# Autodesk Inventor assembly: RailMirrorIrisLens
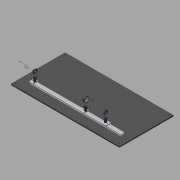
[picture p0: Inventor's stored thumbnail of the model, 180x180]
Saved by Autodesk Inventor 2018 (Build 220112000, 112)
## iProperties
Created: 2018-11-05
Part Number: RailMirrorIrisLens
Document SubType Name: Assembly
Designer: Robert Campbell
Author: Robert Campbell
## Documents named in this file (5)
- \\Mac\Home\Dropbox (UCL - SWC)\work\WorkDocs\MF_BenchOptics\CAD_files\RailMirrorIrisLens.iam
- \\Mac\Home\Dropbox (UCL - SWC)\work\WorkDocs\MF_BenchOptics\CAD_files\RailAndMirror.iam
- \\Mac\Home\Dropbox (UCL - SWC)\work\WorkDocs\MF_BenchOptics\CAD_files\R2_M-Step.ipt
- \\Mac\Home\Dropbox (UCL - SWC)\work\WorkDocs\MF_BenchOptics\CAD_files\LA1256-A-Solidworks.ipt
- \\Mac\Home\Dropbox (UCL - SWC)\work\WorkDocs\MF_BenchOptics\CAD_files\LM2_lensholder_on_mount.iam
## Components (4 placed, 4 different names)
1. RailAndMirror:1 [sub-assembly] — Mate:1, Mate:2, Mate:5, Angle:1
2. R2_M-Step:1 — Mate:1, Mate:2
3. LA1256-A-Solidworks:1 — Mate:3, Mate:4
4. LM2_lensholder_on_mount:1 [sub-assembly] — Mate:3, Mate:4, Mate:5, Angle:1
## Relationships (6: Mate 5, Angle 1)
- Mate:1: RailAndMirror:1 ↔ R2_M-Step:1
- Mate:2: RailAndMirror:1 ↔ R2_M-Step:1
- Mate:3: LA1256-A-Solidworks:1 ↔ LM2_lensholder_on_mount:1
- Mate:4: LA1256-A-Solidworks:1 ↔ LM2_lensholder_on_mount:1
- Mate:5: RailAndMirror:1 ↔ LM2_lensholder_on_mount:1
- Angle:1 (0 deg): RailAndMirror:1 ↔ LM2_lensholder_on_mount:1
